# Autodesk Inventor assembly: Toughbox-mini
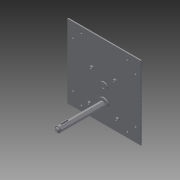
[picture p0: Inventor's stored thumbnail of the model, 180x180]
Saved by Autodesk Inventor 2013 (Build 170138000, 138)
## iProperties
Created: 2013-01-11
Part Number: Toughbox-mini
Document SubType Name: Assembly
Designer: Naphat
Translation Standard: STEP AP203
FileName: S:/Products/Gearboxes Spur Single Stage/Toughbox/Toughbox Mini/Toughbox-Mini.stp
PreProcessor: Unknown
PostProcessor: Build: 138, Release: 2013 RTM - Date: Thu 03/01/2012
Sent Units: millimeter
Uncertainty: 0.001
Author: Naphat
## Documents named in this file (19)
- C:\Autodesk\3.Imported Components\Imported Components\Toughbox-mini\Toughbox-mini.iam
- C:\Autodesk\3.Imported Components\Imported Components\Toughbox-mini\r6zz.ipt
- C:\Autodesk\3.Imported Components\Imported Components\Toughbox-mini\Toughbox_d07.ipt
- C:\Autodesk\3.Imported Components\Imported Components\Toughbox-mini\Toughbox_d05.ipt
- C:\Autodesk\3.Imported Components\Imported Components\Toughbox-mini\Toughbox_d08.ipt
- C:\Autodesk\3.Imported Components\Imported Components\Toughbox-mini\Toughbox_d06.ipt
- C:\Autodesk\3.Imported Components\Imported Components\Toughbox-mini\fr-6-zz.ipt
- C:\Autodesk\3.Imported Components\Imported Components\Toughbox-mini\fr-8-zz.ipt
- C:\Autodesk\3.Imported Components\Imported Components\Toughbox-mini\10-32_nylock_nut.ipt
- C:\Autodesk\3.Imported Components\Imported Components\Toughbox-mini\5-16_washer.ipt
- C:\Autodesk\3.Imported Components\Imported Components\Toughbox-mini\Toughbox_d09.ipt
- C:\Autodesk\3.Imported Components\Imported Components\Toughbox-mini\8mm_spring_clip.ipt
- C:\Autodesk\3.Imported Components\Imported Components\Toughbox-mini\Toughbox-mini_d01-5-12.ipt
- C:\Autodesk\3.Imported Components\Imported Components\Toughbox-mini\250_washer.ipt
- C:\Autodesk\3.Imported Components\Imported Components\Toughbox-mini\14-20x0500_bhcs.ipt
- C:\Autodesk\3.Imported Components\Imported Components\Toughbox-mini\125x124x700_key.ipt
- C:\Autodesk\3.Imported Components\Imported Components\Toughbox-mini\10-32x0625_shcs.ipt
- C:\Autodesk\2.CAD drawing-robot design\Project.1-LDU, 2013 FRC\Components\Hex Shaft.ipt
- C:\Autodesk\2.CAD drawing-robot design\Project.1-LDU, 2013 FRC\Components\Custom GearBox Mount.ipt
## Components (34 placed, 18 different names)
1. r6zz:1
2. r6zz:2
3. Toughbox_d07:1
4. Toughbox_d05:1
5. Toughbox_d08:1
6. Toughbox_d06:1 — Mate:1, Mate:2
7. fr-6-zz:1
8. fr-8-zz:1 — Mate:8
9. 10-32_nylock_nut:1
10. 10-32_nylock_nut:2
11. 10-32_nylock_nut:3
12. 10-32_nylock_nut:4
13. 5-16_washer:1
14. 5-16_washer:2
15. 5-16_washer:3
16. 5-16_washer:4
17. Toughbox_d09:1
18. Toughbox_d09:2
19. 8mm_spring_clip:1
20. 8mm_spring_clip:2
21. Toughbox-mini_d01-5-12:1 — Mate:3, Mate:7
22. 250_washer:1 — Mate:4, Mate:5
23. 14-20x0500_bhcs:1 — Mate:4, Mate:5
24. 125x124x700_key:1 — Mate:6
25. 10-32x0625_shcs:1
26. 10-32x0625_shcs:2
27. 10-32x0625_shcs:3
28. 10-32x0625_shcs:4
29. 10-32x0625_shcs:5
30. 10-32x0625_shcs:6
31. 10-32x0625_shcs:7
32. 10-32x0625_shcs:8
33. Hex Shaft:1 — Mate:1, Mate:2, Mate:3, Mate:6
34. Custom GearBox Mount:1 — Mate:7, Mate:8
## Relationships (8: Mate 8)
- Mate:1: Toughbox_d06:1 ↔ Hex Shaft:1
- Mate:2: Toughbox_d06:1 ↔ Hex Shaft:1
- Mate:3: Toughbox-mini_d01-5-12:1 ↔ Hex Shaft:1
- Mate:4: 250_washer:1 ↔ 14-20x0500_bhcs:1
- Mate:5: 250_washer:1 ↔ 14-20x0500_bhcs:1
- Mate:6: 125x124x700_key:1 ↔ Hex Shaft:1
- Mate:7: Toughbox-mini_d01-5-12:1 ↔ Custom GearBox Mount:1
- Mate:8: fr-8-zz:1 ↔ Custom GearBox Mount:1
